# Autodesk Inventor assembly: TOF_Z_GOLDPIANMI
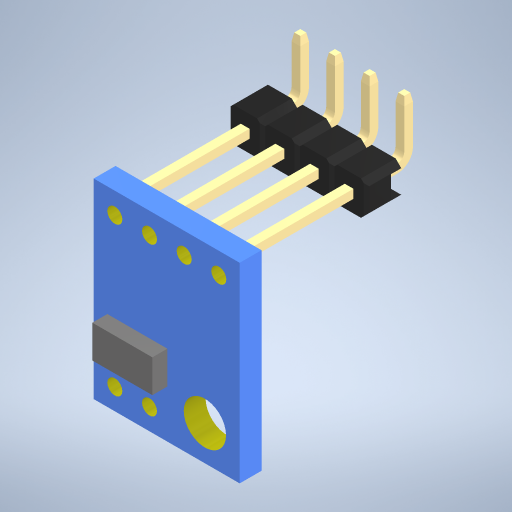
[picture p0: Inventor's stored thumbnail of the model, 512x512]
Saved by Autodesk Inventor 2023 (Build 270158000, 158)
## iProperties
Created: 2024-05-14
Part Number: TOF_Z_GOLDPIANMI
Document SubType Name: Assembly
Designer: kamil
Author: kamil
## Documents named in this file (3)
- C:\Users\kamil\Documents\PROJECTS - repos\ModBot---Projekt-Zespolowy\mechanics\TOF_Z_GOLDPIANMI.iam
- C:\Users\kamil\Documents\PROJECTS - repos\ModBot---Projekt-Zespolowy\mechanics\1x4 Male Pin Header Angle.ipt
- C:\Users\kamil\Documents\PROJECTS - repos\ModBot---Projekt-Zespolowy\mechanics\TOF_VL53L0X (1).ipt
## Components (2 placed, 2 different names)
1. 1x4 Male Pin Header Angle:1 — Równoległe:1, Zestawiające:1, Równoległe:2
2. TOF_VL53L0X (1):1 — Równoległe:1, Zestawiające:1, Równoległe:2
## Relationships (3: Flush 2, Mate 1)
- Równoległe:1 [Flush] (-0.27 mm): 1x4 Male Pin Header Angle:1 ↔ TOF_VL53L0X (1):1
- Zestawiające:1 [Mate] (8.5 mm): 1x4 Male Pin Header Angle:1 ↔ TOF_VL53L0X (1):1
- Równoległe:2 [Flush] (-0.3 mm): 1x4 Male Pin Header Angle:1 ↔ TOF_VL53L0X (1):1
